# Autodesk Inventor assembly: rigt_motor_asembly
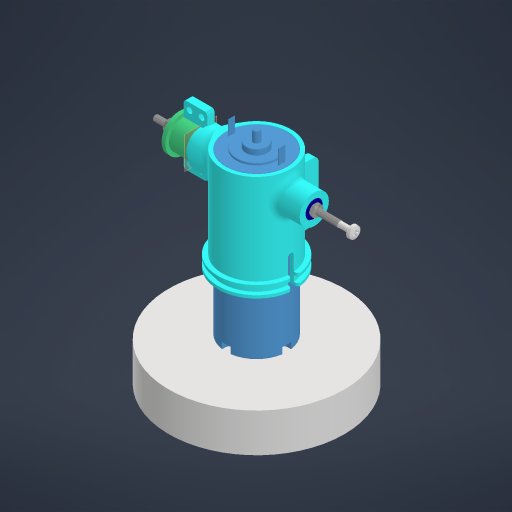
[picture p0: Inventor's stored thumbnail of the model, 512x512]
Saved by Autodesk Inventor 2024 (Build 280153000, 153)
## iProperties
Created: 2023-05-14
Part Number: rigt_motor_asembly
Document SubType Name: Assembly
Designer: user
Author: user
## Documents named in this file (8)
- D:\Docs\Robot\3d\motor_assembly\rigt_motor_asembly.iam
- D:\Docs\Robot\3d\motor_assembly\rigt_motor_asembly\lower_arm.ipt
- D:\Docs\Robot\3d\motor_assembly\bushing_assembly.iam
- D:\Docs\Robot\3d\default_components\motor.ipt
- D:\Docs\Robot\3d\default_components\wheel.ipt
- D:\Docs\Robot\3d\default_components\604zz_bearing.ipt
- C:\Users\user\Documents\Inventor\Content Center Files\R2024\ru-RU\DIN 934\DIN 934 - M4 x 0,7.ipt
- C:\Users\user\Documents\Inventor\Content Center Files\R2024\ru-RU\DIN 7985 (H)\DIN 7985 (H) - M4x30-H.ipt
## Components (7 placed, 7 different names)
1. lower_arm:1 — Совмещение:1, Совмещение:2, Совмещение:3, Совмещение:4, Вставка:5, Вставка:6, Вставка:7, Заподлицо:1
2. bushing_assembly:2 [sub-assembly] — Вставка:6, Заподлицо:1
3. motor:1 — Вставка:4, Вставка:5
4. wheel:1 — Вставка:4
5. 604zz_bearing:1 — Вставка:7, Вставка:8, Вставка:11
6. DIN 934 - заменено на DIN EN 24032/28673/28674 M4:1 — Вставка:8
7. DIN 7985 (H) M4x30-H:1 — Вставка:11
## Relationships (11: Insert 6, Mate 4, Flush 1)
- Совмещение:1 [Mate]: lower_arm:1
- Совмещение:2 [Mate]: lower_arm:1
- Совмещение:3 [Mate]: lower_arm:1
- Вставка:4 [Insert]: motor:1 ↔ wheel:1
- Совмещение:4 [Mate]: lower_arm:1
- Вставка:5 [Insert]: lower_arm:1 ↔ motor:1
- Вставка:6 [Insert]: lower_arm:1 ↔ bushing_assembly:2
- Вставка:7 [Insert]: lower_arm:1 ↔ 604zz_bearing:1
- Вставка:8 [Insert]: 604zz_bearing:1 ↔ DIN 934 - заменено на DIN EN 24032/28673/28674 M4:1
- Вставка:11 [Insert]: 604zz_bearing:1 ↔ DIN 7985 (H) M4x30-H:1
- Заподлицо:1 [Flush]: lower_arm:1 ↔ bushing_assembly:2
